# Autodesk Inventor assembly: CanSat
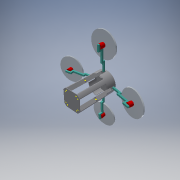
[picture p0: Inventor's stored thumbnail of the model, 180x180]
Saved by Autodesk Inventor 2018 (Build 220112000, 112)
## iProperties
Created: 2017-12-31
Part Number: CanSat
Document SubType Name: Assembly
Designer: suchanek
Author: suchanek
## Documents named in this file (7)
- C:\Users\sucha\programming\CanSat\Schematics\Model\CanSat.iam
- C:\Users\sucha\programming\CanSat\Schematics\Model\Hull.ipt
- C:\Users\sucha\programming\CanSat\Schematics\Model\Arm.ipt
- C:\Users\sucha\programming\CanSat\Schematics\Model\Flight_controler.ipt
- C:\Users\sucha\programming\CanSat\Schematics\Model\Motor.ipt
- C:\Users\sucha\programming\CanSat\Schematics\Model\Rotor.ipt
- C:\Users\sucha\programming\CanSat\Schematics\Model\Battery_small.ipt
## Components (30 placed, 6 different names)
1. Hull:1 — Rigid:1, Rotational:4, Rotational:5, Rotational:6, Rotational:7, Cylindrical:1, Mate:2, Mate:3, Mate:13, Mate:14, Mate:15, Cylindrical:2, Mate:16, Mate:17, Mate:18, Mate:19, Mate:20
2. Arm:1 — Rotational:5, Rigid:5
3. Arm:2 — Rotational:4, Rigid:4
4. Arm:3 — Rotational:7, Rigid:3
5. Arm:4 — Rotational:6, Rigid:2
6. Flight_controler:1 — Rigid:1
7. Motor:1 — Rigid:2, Rotational:8
8. Motor:2 — Rigid:3, Rotational:9
9. Motor:3 — Rigid:4, Rotational:11
10. Motor:4 — Rigid:5, Rotational:10
11. Rotor:1 — Rotational:8
12. Rotor:2 — Rotational:10
13. Rotor:3 — Rotational:9
14. Rotor:4 — Rotational:11
15. Battery_small:1 — Cylindrical:1, Rotational:12, Mate:1, Mate:2, Rotational:13
16. Battery_small:2 — Rotational:12, Mate:1
17. Battery_small:3 — Rotational:13, Mate:3, Rotational:14, Mate:4
18. Battery_small:4 — Rotational:18, Mate:9, Rotational:22, Cylindrical:2
19. Battery_small:5 — Rotational:18, Mate:9
20. Battery_small:6 — Rotational:17, Mate:7, Mate:11
21. Battery_small:7 — Rotational:14, Mate:4
22. Battery_small:8 — Rotational:16, Mate:6, Mate:12
23. Battery_small:9 — Rotational:19, Mate:8
24. Battery_small:10 — Rotational:19, Mate:8, Rotational:23, Mate:19, Mate:20
25. Battery_small:11 — Rotational:20, Mate:10, Rotational:23, Mate:18
26. Battery_small:12 — Rotational:20, Mate:10
27. Battery_small:13 — Mate:5, Rotational:15
28. Battery_small:14 — Rotational:17, Mate:7, Mate:11, Rotational:22, Mate:16, Mate:17
29. Battery_small:15 — Mate:5, Rotational:15, Rotational:21, Mate:15
30. Battery_small:16 — Rotational:16, Mate:6, Mate:12, Rotational:21, Mate:13, Mate:14
## Relationships (47: RevoluteJoint 20, Mate 20, WeldJoint 5, CylindricalJoint 2)
- Rigid:1 [WeldJoint]: Hull:1 ↔ Flight_controler:1
- Rotational:4 [RevoluteJoint]: Hull:1 ↔ Arm:2
- Rotational:5 [RevoluteJoint]: Hull:1 ↔ Arm:1
- Rotational:6 [RevoluteJoint]: Hull:1 ↔ Arm:4
- Rotational:7 [RevoluteJoint]: Hull:1 ↔ Arm:3
- Rigid:2 [WeldJoint]: Arm:4 ↔ Motor:1
- Rotational:8 [RevoluteJoint]: Motor:1 ↔ Rotor:1
- Rigid:3 [WeldJoint]: Arm:3 ↔ Motor:2
- Rotational:9 [RevoluteJoint]: Motor:2 ↔ Rotor:3
- Rigid:4 [WeldJoint]: Arm:2 ↔ Motor:3
- Rigid:5 [WeldJoint]: Arm:1 ↔ Motor:4
- Rotational:10 [RevoluteJoint]: Motor:4 ↔ Rotor:2
- Rotational:11 [RevoluteJoint]: Motor:3 ↔ Rotor:4
- Cylindrical:1: Hull:1 ↔ Battery_small:1
- Rotational:12 [RevoluteJoint] (5 mm): Battery_small:1 ↔ Battery_small:2
- Mate:1: Battery_small:1 ↔ Battery_small:2
- Mate:2: Hull:1 ↔ Battery_small:1
- Rotational:13 [RevoluteJoint]: Battery_small:1 ↔ Battery_small:3
- Mate:3: Hull:1 ↔ Battery_small:3
- Rotational:14 [RevoluteJoint] (5 mm): Battery_small:3 ↔ Battery_small:7
- Mate:4: Battery_small:3 ↔ Battery_small:7
- Mate:5: Battery_small:13 ↔ Battery_small:15
- Rotational:15 [RevoluteJoint] (5 mm): Battery_small:13 ↔ Battery_small:15
- Rotational:16 [RevoluteJoint] (5 mm): Battery_small:8 ↔ Battery_small:16
- Rotational:17 [RevoluteJoint] (5 mm): Battery_small:6 ↔ Battery_small:14
- Rotational:18 [RevoluteJoint] (5 mm): Battery_small:4 ↔ Battery_small:5
- Rotational:19 [RevoluteJoint] (5 mm): Battery_small:9 ↔ Battery_small:10
- Mate:6: Battery_small:8 ↔ Battery_small:16
- Mate:7: Battery_small:6 ↔ Battery_small:14
- Rotational:20 [RevoluteJoint] (5 mm): Battery_small:11 ↔ Battery_small:12
- Mate:8: Battery_small:9 ↔ Battery_small:10
- Mate:9: Battery_small:4 ↔ Battery_small:5
- Mate:10: Battery_small:11 ↔ Battery_small:12
- Mate:11: Battery_small:6 ↔ Battery_small:14
- Mate:12: Battery_small:8 ↔ Battery_small:16
- Rotational:21 [RevoluteJoint]: Battery_small:15 ↔ Battery_small:16
- Rotational:22 [RevoluteJoint]: Battery_small:4 ↔ Battery_small:14
- Rotational:23 [RevoluteJoint]: Battery_small:10 ↔ Battery_small:11
- Mate:13: Hull:1 ↔ Battery_small:16
- Mate:14: Hull:1 ↔ Battery_small:16
- Mate:15: Hull:1 ↔ Battery_small:15
- Cylindrical:2: Hull:1 ↔ Battery_small:4
- Mate:16: Hull:1 ↔ Battery_small:14
- Mate:17: Hull:1 ↔ Battery_small:14
- Mate:18: Hull:1 ↔ Battery_small:11
- Mate:19: Hull:1 ↔ Battery_small:10
- Mate:20: Hull:1 ↔ Battery_small:10
